# Autodesk Inventor assembly: Pi_Camera_Mount_Assembly
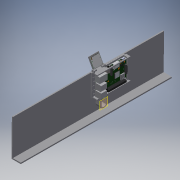
[picture p0: Inventor's stored thumbnail of the model, 180x180]
Saved by Autodesk Inventor 2017 (Build 210142000, 142)
## iProperties
Created: 2020-02-20
Part Number: Pi_Camera_Mount_Assembly
Document SubType Name: Assembly
Designer: S346553810
Author: S346553810
## Documents named in this file (6)
- \\ad.ocdsb.ca\studenthome\3\S338674153\FRC 2020\FullRobotRefactor\Camera\Pi_Camera_Mount_Assembly.iam
- \\ad.ocdsb.ca\studenthome\3\S338674153\FRC 2020\FullRobotRefactor\Camera\Pi_Camera_Crossbar_Mount.ipt
- \\ad.ocdsb.ca\studenthome\3\S338674153\FRC 2020\FullRobotRefactor\Camera\PI_Box_FINAL_COPY2.ipt
- \\ad.ocdsb.ca\studenthome\3\S338674153\FRC 2020\FullRobotRefactor\Camera\Top of the cam case (real version).ipt
- \\ad.ocdsb.ca\studenthome\3\S338674153\FRC 2020\FullRobotRefactor\Camera\Rpi3Bplus.ipt
- \\ad.ocdsb.ca\studenthome\3\S338674153\FRC 2020\FullRobotRefactor\Camera\RasPi_Camera.ipt
## Components (5 placed, 5 different names)
1. Pi_Camera_Crossbar_Mount:1 — Mate:1, Flush:1, Mate:2
2. PI_Box_FINAL_COPY2:1 — Mate:1, Flush:1, Mate:2, Mate:3, Mate:4, Angle:1, Mate:7, Mate:8, Mate:9
3. Top of the cam case (real version):1 — Mate:3, Mate:4, Mate:5, Mate:6
4. Rpi3Bplus:1 — Angle:1, Mate:7, Mate:8, Mate:9
5. RasPi_Camera:1 — Mate:5, Mate:6
## Relationships (11: Mate 9, Flush 1, Angle 1)
- Mate:1: Pi_Camera_Crossbar_Mount:1 ↔ PI_Box_FINAL_COPY2:1
- Flush:1: Pi_Camera_Crossbar_Mount:1 ↔ PI_Box_FINAL_COPY2:1
- Mate:2 (234.95 mm): Pi_Camera_Crossbar_Mount:1 ↔ PI_Box_FINAL_COPY2:1
- Mate:3: PI_Box_FINAL_COPY2:1 ↔ Top of the cam case (real version):1
- Mate:4: PI_Box_FINAL_COPY2:1 ↔ Top of the cam case (real version):1
- Mate:5: Top of the cam case (real version):1 ↔ RasPi_Camera:1
- Mate:6: Top of the cam case (real version):1 ↔ RasPi_Camera:1
- Angle:1 (0 deg): PI_Box_FINAL_COPY2:1 ↔ Rpi3Bplus:1
- Mate:7: PI_Box_FINAL_COPY2:1 ↔ Rpi3Bplus:1
- Mate:8: PI_Box_FINAL_COPY2:1 ↔ Rpi3Bplus:1
- Mate:9: PI_Box_FINAL_COPY2:1 ↔ Rpi3Bplus:1
